# Autodesk Inventor assembly: default_motor_asembly
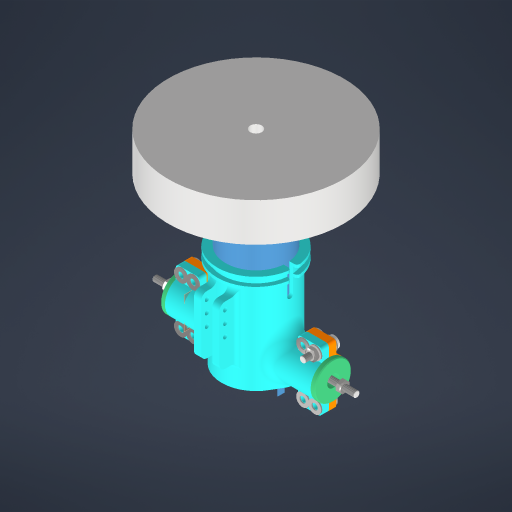
[picture p0: Inventor's stored thumbnail of the model, 512x512]
Saved by Autodesk Inventor 2024 (Build 280153000, 153)
## iProperties
Created: 2023-05-13
Part Number: default_motor_asembly
Document SubType Name: Assembly
Designer: user
Author: user
## Documents named in this file (9)
- D:\Docs\Robot\3d\motor_assembly\default_motor_asembly.iam
- D:\Docs\Robot\3d\motor_assembly\default_motor_asembly\lower_arm.ipt
- D:\Docs\Robot\3d\motor_assembly\bushing_assembly.iam
- D:\Docs\Robot\3d\default_components\motor.ipt
- C:\Users\user\Documents\Inventor\Content Center Files\R2024\ru-RU\DIN 125-1  A\DIN 125 - A 4,3.ipt
- C:\Users\user\Documents\Inventor\Content Center Files\R2024\ru-RU\DIN 7985 (H)\DIN 7985 (H) - M4x20-H.ipt
- C:\Users\user\Documents\Inventor\Content Center Files\R2024\ru-RU\DIN 934\DIN 934 - M4 x 0,7.ipt
- D:\Docs\Robot\3d\default_components\wheel.ipt
- D:\Docs\Robot\3d\motor_assembly\default_motor_asembly\cup.ipt
## Components (25 placed, 8 different names)
1. lower_arm:1 — Совмещение:1, Совмещение:2, Совмещение:3, Вставка:2, Вставка:5, Вставка:6, Совмещение:4, Вставка:7, Вставка:8, Вставка:13, Вставка:14, Вставка:15, Вставка:16, Заподлицо:1, Заподлицо:3, Вставка:28, Вставка:29
2. bushing_assembly:1 [sub-assembly] — Заподлицо:2, Заподлицо:3
3. bushing_assembly:2 [sub-assembly] — Вставка:2
4. motor:1 — Вставка:5, Вставка:23
5. DIN 125-1 A A 4,3:1 — Вставка:6
6. DIN 125-1 A A 4,3:2 — Совмещение:4
7. DIN 125-1 A A 4,3:3 — Вставка:8
8. DIN 125-1 A A 4,3:4 — Вставка:7
9. DIN 125-1 A A 4,3:5 — Вставка:24
10. DIN 125-1 A A 4,3:6 — Вставка:26
11. DIN 125-1 A A 4,3:7 — Вставка:27
12. DIN 125-1 A A 4,3:8 — Вставка:25
13. DIN 125-1 A A 4,3:9 — Вставка:13, Вставка:22
14. DIN 125-1 A A 4,3:10 — Вставка:14
15. DIN 125-1 A A 4,3:11 — Вставка:15
16. DIN 125-1 A A 4,3:12 — Вставка:16
17. DIN 125-1 A A 4,3:13 — Вставка:30
18. DIN 125-1 A A 4,3:14 — Вставка:31
19. DIN 125-1 A A 4,3:15 — Вставка:32
20. DIN 125-1 A A 4,3:16 — Вставка:21, Вставка:33
21. DIN 7985 (H) M4x20-H:1 — Вставка:21
22. DIN 934 - заменено на DIN EN 24032/28673/28674 M4:1 — Вставка:22
23. wheel:1 — Вставка:23
24. cup:1 — Заподлицо:1, Заподлицо:2, Вставка:24, Вставка:25, Вставка:26, Вставка:27
25. cup:2 — Вставка:28, Вставка:29, Вставка:30, Вставка:31, Вставка:32, Вставка:33
## Relationships (29: Insert 22, Mate 4, Flush 3)
- Совмещение:1 [Mate]: lower_arm:1
- Совмещение:2 [Mate]: lower_arm:1
- Совмещение:3 [Mate]: lower_arm:1
- Вставка:2 [Insert]: lower_arm:1 ↔ bushing_assembly:2
- Вставка:5 [Insert]: lower_arm:1 ↔ motor:1
- Вставка:6 [Insert]: lower_arm:1 ↔ DIN 125-1 A A 4,3:1
- Совмещение:4 [Mate]: lower_arm:1 ↔ DIN 125-1 A A 4,3:2
- Вставка:7 [Insert]: lower_arm:1 ↔ DIN 125-1 A A 4,3:4
- Вставка:8 [Insert]: lower_arm:1 ↔ DIN 125-1 A A 4,3:3
- Вставка:13 [Insert]: lower_arm:1 ↔ DIN 125-1 A A 4,3:9
- Вставка:14 [Insert]: lower_arm:1 ↔ DIN 125-1 A A 4,3:10
- Вставка:15 [Insert]: lower_arm:1 ↔ DIN 125-1 A A 4,3:11
- Вставка:16 [Insert]: lower_arm:1 ↔ DIN 125-1 A A 4,3:12
- Вставка:21 [Insert]: DIN 125-1 A A 4,3:16 ↔ DIN 7985 (H) M4x20-H:1
- Вставка:22 [Insert]: DIN 125-1 A A 4,3:9 ↔ DIN 934 - заменено на DIN EN 24032/28673/28674 M4:1
- Вставка:23 [Insert]: motor:1 ↔ wheel:1
- Заподлицо:1 [Flush]: lower_arm:1 ↔ cup:1
- Заподлицо:2 [Flush]: bushing_assembly:1 ↔ cup:1
- Вставка:24 [Insert]: DIN 125-1 A A 4,3:5 ↔ cup:1
- Вставка:25 [Insert]: DIN 125-1 A A 4,3:8 ↔ cup:1
- Вставка:26 [Insert]: DIN 125-1 A A 4,3:6 ↔ cup:1
- Вставка:27 [Insert]: DIN 125-1 A A 4,3:7 ↔ cup:1
- Заподлицо:3 [Flush]: lower_arm:1 ↔ bushing_assembly:1
- Вставка:28 [Insert]: lower_arm:1 ↔ cup:2
- Вставка:29 [Insert]: lower_arm:1 ↔ cup:2
- Вставка:30 [Insert]: DIN 125-1 A A 4,3:13 ↔ cup:2
- Вставка:31 [Insert]: DIN 125-1 A A 4,3:14 ↔ cup:2
- Вставка:32 [Insert]: DIN 125-1 A A 4,3:15 ↔ cup:2
- Вставка:33 [Insert]: DIN 125-1 A A 4,3:16 ↔ cup:2
